# Autodesk Inventor assembly: myrobot
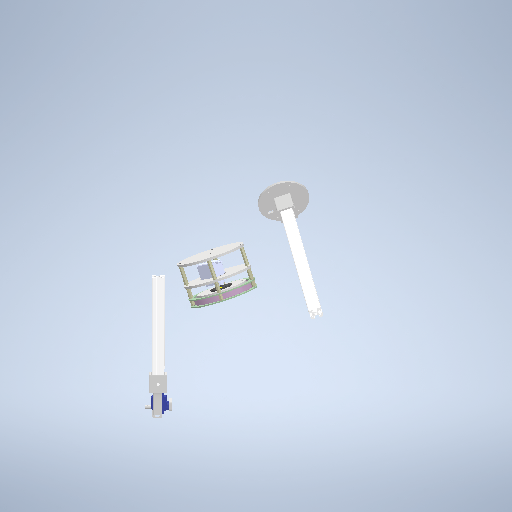
[picture p0: Inventor's stored thumbnail of the model, 512x512]
Saved by Autodesk Inventor 2025 (Build 290162000, 162)
## iProperties
Created: 2024-05-26
Part Number: myrobot
Document SubType Name: Assembly
Designer: hifzh
Author: hifzh
## Documents named in this file (18)
- C:\Users\hifzhil\final_year\Design\TA-Design\part\myrobot - v0.iam
- C:\Users\hifzhil\final_year\Design\TA-Design\part\Base_link\lower-plate.ipt
- C:\Users\hifzhil\final_year\Design\TA-Design\part\Base_link\6815RS Bearing v1\6815RS Bearing.iam
- C:\Users\hifzhil\final_year\Design\TA-Design\part\Base_link\Ring Plate v1.ipt
- C:\Users\hifzhil\final_year\Design\TA-Design\part\Base_link\M3x10mm Hex Standoff v1.ipt
- C:\Users\hifzhil\final_year\Design\TA-Design\part\Base_link\M3x32mm Hex Standoff v1.ipt
- C:\Users\hifzhil\final_year\Design\TA-Design\part\servo-holder3.ipt
- C:\Users\hifzhil\final_year\Design\TA-Design\part\almini-18cm.ipt
- C:\Users\hifzhil\final_year\Design\TA-Design\part\almini-26cm.ipt
- C:\Users\hifzhil\final_year\Design\TA-Design\part\Base_link\M3x19mm Hex Standoff v1.ipt
- C:\Users\hifzhil\final_year\Design\TA-Design\part\Base_link\clip_mount.ipt
- C:\Users\hifzhil\final_year\Design\TA-Design\part\lower-plate-sg90.ipt
- C:\Users\hifzhil\final_year\Design\TA-Design\part\Base_link\bottom-plate.ipt
- C:\Users\hifzhil\final_year\Design\TA-Design\part\servos.ipt
- C:\Users\hifzhil\final_year\Design\TA-Design\part\futaba_horn_35mm_round v1.ipt
- C:\Users\hifzhil\final_year\Design\TA-Design\part\SG90 v2.ipt
- C:\Users\hifzhil\final_year\Design\TA-Design\part\SG90-horn v1.ipt
- C:\Users\hifzhil\final_year\Design\TA-Design\part\end-effector.ipt
## Components (31 placed, 17 different names)
1. lower-plate:1 — Insert:9, Insert:10, Insert:11, Insert:12, Rigid:8
2. 6815RS Bearing:1 [sub-assembly] — Mate:7, Rigid:7, Rigid:8
3. Ring Plate v1:1 — Mate:7, Insert:3, Insert:4, Insert:5, Insert:6, Rigid:7, Insert:37, Insert:38, Insert:39, Insert:40
4. Ring Plate v1:2 — Insert:7, Insert:8
5. M3x10mm Hex Standoff v1:1 — Insert:3, Insert:8
6. M3x10mm Hex Standoff v1:2 — Insert:4, Insert:7
7. M3x10mm Hex Standoff v1:3 — Insert:6
8. M3x10mm Hex Standoff v1:4 — Insert:5
9. M3x10mm Hex Standoff v1:5 — Insert:9
10. M3x10mm Hex Standoff v1:6 — Insert:10
11. M3x10mm Hex Standoff v1:7 — Insert:11
12. M3x10mm Hex Standoff v1:8 — Insert:12
13. servo-holder3:1 — Rigid:11, Insert:63, Insert:64
14. almini-18cm:1 — Rigid:11
15. almini-26cm:1 — Rigid:12
16. M3x19mm Hex Standoff v1:1 — Insert:40
17. M3x19mm Hex Standoff v1:2 — Insert:39, Insert:62
18. M3x19mm Hex Standoff v1:3 — Insert:38, Insert:61
19. M3x19mm Hex Standoff v1:4 — Insert:37
20. M3x32mm Hex Standoff v1:1 — Insert:56, Insert:59
21. M3x32mm Hex Standoff v1:2 — Insert:55
22. M3x32mm Hex Standoff v1:3 — Insert:48
23. M3x32mm Hex Standoff v1:4 — Insert:47, Insert:60
24. clip_mount:1 — Insert:47, Insert:48, Insert:55, Insert:56
25. lower-plate-sg90:2 — Rigid:12
26. bottom-plate:1 — Insert:57, Insert:58, Insert:59, Insert:60, Insert:61, Insert:62
27. servos:1 — Insert:57, Insert:58, Rotational:7
28. futaba_horn_35mm_round v1:1 — Rotational:7
29. SG90 v2:1 — Insert:63, Insert:64, Rotational:8
30. SG90-horn v1:1 — Rotational:8, Insert:65, Insert:66
31. end-effector:1 — Insert:65, Insert:66
## Relationships (35: Insert 28, WeldJoint 4, RevoluteJoint 2, Mate 1)
- Mate:7: 6815RS Bearing:1 ↔ Ring Plate v1:1
- Insert:3: Ring Plate v1:1 ↔ M3x10mm Hex Standoff v1:1
- Insert:4: Ring Plate v1:1 ↔ M3x10mm Hex Standoff v1:2
- Insert:5: Ring Plate v1:1 ↔ M3x10mm Hex Standoff v1:4
- Insert:6: Ring Plate v1:1 ↔ M3x10mm Hex Standoff v1:3
- Rigid:7 [WeldJoint] (10 mm): 6815RS Bearing:1 ↔ Ring Plate v1:1
- Insert:7: Ring Plate v1:2 ↔ M3x10mm Hex Standoff v1:2
- Insert:8: Ring Plate v1:2 ↔ M3x10mm Hex Standoff v1:1
- Insert:9: lower-plate:1 ↔ M3x10mm Hex Standoff v1:5
- Insert:10: lower-plate:1 ↔ M3x10mm Hex Standoff v1:6
- Insert:11: lower-plate:1 ↔ M3x10mm Hex Standoff v1:7
- Insert:12: lower-plate:1 ↔ M3x10mm Hex Standoff v1:8
- Rigid:8 [WeldJoint]: lower-plate:1 ↔ 6815RS Bearing:1
- Rigid:11 [WeldJoint]: servo-holder3:1 ↔ almini-18cm:1
- Insert:37: Ring Plate v1:1 ↔ M3x19mm Hex Standoff v1:4
- Insert:38: Ring Plate v1:1 ↔ M3x19mm Hex Standoff v1:3
- Insert:39: Ring Plate v1:1 ↔ M3x19mm Hex Standoff v1:2
- Insert:40: Ring Plate v1:1 ↔ M3x19mm Hex Standoff v1:1
- Insert:47: M3x32mm Hex Standoff v1:4 ↔ clip_mount:1
- Insert:48: M3x32mm Hex Standoff v1:3 ↔ clip_mount:1
- Insert:55: M3x32mm Hex Standoff v1:2 ↔ clip_mount:1
- Insert:56: M3x32mm Hex Standoff v1:1 ↔ clip_mount:1
- Rigid:12 [WeldJoint]: almini-26cm:1 ↔ lower-plate-sg90:2
- Insert:57: bottom-plate:1 ↔ servos:1
- Insert:58: bottom-plate:1 ↔ servos:1
- Insert:59: M3x32mm Hex Standoff v1:1 ↔ bottom-plate:1
- Insert:60: M3x32mm Hex Standoff v1:4 ↔ bottom-plate:1
- Rotational:7 [RevoluteJoint]: servos:1 ↔ futaba_horn_35mm_round v1:1
- Insert:61: M3x19mm Hex Standoff v1:3 ↔ bottom-plate:1
- Insert:62: M3x19mm Hex Standoff v1:2 ↔ bottom-plate:1
- Insert:63: servo-holder3:1 ↔ SG90 v2:1
- Insert:64: servo-holder3:1 ↔ SG90 v2:1
- Rotational:8 [RevoluteJoint]: SG90 v2:1 ↔ SG90-horn v1:1
- Insert:65: SG90-horn v1:1 ↔ end-effector:1
- Insert:66: SG90-horn v1:1 ↔ end-effector:1
